# Autodesk Inventor assembly: BRcA_2_with_microphone_plug
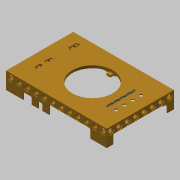
[picture p0: Inventor's stored thumbnail of the model, 180x180]
Saved by Autodesk Inventor 2019.3 (Build 233278000, 278)
## iProperties
Created: 2019-04-11
Part Number: BRcA_2_with_microphone_plug
Document SubType Name: Assembly
Designer: Varga Daniel
Author: Varga Daniel
## Documents named in this file (3)
- C:\!_Dani\!_cloud\OneDrive\!_munka\Revolution\RevvyDemoKit\Structural parts\Demonstrations\Kickstarter videos\Brain pcb\BRcA_2_with_microphone_plug.iam
- C:\!_Dani\!_cloud\OneDrive\!_munka\Revolution\RevvyDemoKit\Structural parts\Demonstrations\Kickstarter videos\Brain pcb\BRcA_2.ipt
- C:\!_Dani\!_cloud\OneDrive\!_munka\Revolution\RevvyDemoKit\Structural parts\Demonstrations\Kickstarter videos\Brain pcb\Microphone_hole_plug.ipt
## Components (2 placed, 2 different names)
1. BRcA_2:1 — Flush:1, Mate:1, Mate:2
2. Microphone_hole_plug:1 — Flush:1, Mate:1, Mate:2
## Relationships (3: Mate 2, Flush 1)
- Flush:1: BRcA_2:1 ↔ Microphone_hole_plug:1
- Mate:1: BRcA_2:1 ↔ Microphone_hole_plug:1
- Mate:2: BRcA_2:1 ↔ Microphone_hole_plug:1
